# Autodesk Inventor assembly: E-AXIS ASSEMBLY
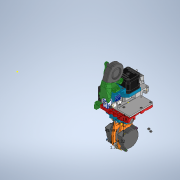
[picture p0: Inventor's stored thumbnail of the model, 180x180]
Saved by Autodesk Inventor 2020 (Build 240168000, 168)
## iProperties
Created: 2019-09-18
Part Number: E-AXIS ASSEMBLY
Document SubType Name: Assembly
Designer: pepd9
Author: pepd9
## Documents named in this file (43)
- C:\DESIGNS\MK3PRO P1\E-Axis\E-AXIS ASSEMBLY.iam
- C:\DESIGNS\MK3PRO P1\COMPONENTS\LM10UU.ipt
- C:\DESIGNS\MK3PRO P1\E-Axis\X-Carriage V1.3.ipt
- C:\DESIGNS\MK3PRO P1\COMPONENTS\M3 Nut.ipt
- C:\DESIGNS\MK3PRO P1\COMPONENTS\SHCS_M3_10.ipt
- C:\DESIGNS\MK3PRO P1\COMPONENTS\SHCS_M3_40.ipt
- C:\DESIGNS\MK3PRO P1\COMPONENTS\NUT_SQUARE_M3.ipt
- C:\DESIGNS\MK3PRO P1\E-Axis\Extruder_stepper_motor.iam
- C:\DESIGNS\MK3PRO P1\COMPONENTS\Bondtech Idler.ipt
- C:\DESIGNS\MK3PRO P1\COMPONENTS\Bondtech Driver.ipt
- C:\DESIGNS\MK3PRO P1\COMPONENTS\SHCS_M3_12.ipt
- C:\DESIGNS\MK3PRO P1\E-Axis\x-Carriage Backplate V1.2.ipt
- C:\DESIGNS\MK3PRO P1\COMPONENTS\SHCS_M3_18.ipt
- C:\DESIGNS\MK3PRO P1\E-Axis\E3D_V6.ipt
- C:\DESIGNS\MK3PRO P1\E-Axis\PINDA_Probe.ipt
- C:\DESIGNS\MK3PRO P1\COMPONENTS\Noctua-NF-A4x10.ipt
- C:\DESIGNS\MK3PRO P1\E-Axis\extruder-cover.ipt
- C:\DESIGNS\MK3PRO P1\E-Axis\Fan Support Front.ipt
- C:\DESIGNS\MK3PRO P1\COMPONENTS\SHCS_M3_8.ipt
- C:\DESIGNS\MK3PRO P1\COMPONENTS\SHCS_M3_20.ipt
- C:\DESIGNS\MK3PRO P1\COMPONENTS\SHCS_M3_14.ipt
- C:\DESIGNS\MK3PRO P1\E-Axis\Endstop Trigger Block.ipt
- C:\DESIGNS\MK3PRO P1\E-Axis\Extruder Back V2.ipt
- C:\DESIGNS\MK3PRO P1\E-Axis\Extruder Idler V2.ipt
- C:\DESIGNS\MK3PRO P1\COMPONENTS\M3 Washer.ipt
- C:\DESIGNS\MK3PRO P1\E-Axis\Front Left FanShrowd V1.0.ipt
- C:\DESIGNS\MK3PRO P1\E-Axis\Left Cable Guide.ipt
- C:\DESIGNS\MK3PRO P1\E-Axis\Teflon Placeholder.ipt
- C:\DESIGNS\MK3PRO P1\COMPONENTS\Small Limit Switch\Small Limit Switch.iam
- C:\DESIGNS\MK3PRO P1\COMPONENTS\SHCS_M3_30.ipt
- C:\DESIGNS\MK3PRO P1\COMPONENTS\SHCS_M3_35.ipt
- C:\DESIGNS\MK3PRO P1\E-Axis\E-Motor Mount P1.1.ipt
- C:\DESIGNS\MK3PRO P1\E-Axis\Extruder Cable Clamp.ipt
- C:\DESIGNS\MK3PRO P1\E-Axis\LimitSwitch Container.ipt
- C:\DESIGNS\MK3PRO P1\E-Axis\LimitSwitch Con Lid.ipt
- C:\DESIGNS\MK3PRO P1\COMPONENTS\FAN_5015_BLOWER.ipt
- C:\DESIGNS\MK3PRO P1\E-Axis\Rear Fan Backplate Mount.ipt
- C:\DESIGNS\MK3PRO P1\E-Axis\Rear Left Fan Cover.ipt
- C:\DESIGNS\MK3PRO P1\E-Axis\Rear Left Fan Mount.ipt
- C:\DESIGNS\MK3PRO P1\E-Axis\Rear Right Fan Mount.ipt
- C:\DESIGNS\MK3PRO P1\E-Axis\Rear Cable Clamp.ipt
- C:\DESIGNS\MK3PRO P1\COMPONENTS\SHCS_M3_25.ipt
- C:\DESIGNS\MK3PRO P1\E-Axis\Rear Cable Clamp1.ipt
## Components (107 placed, 42 different names)
1. LM10UU:1 — Mate:1, Mate:2, Mate:5
2. LM10UU:2 — Mate:1, Mate:3, Mate:6
3. LM10UU:3 — Mate:4, Mate:7
4. X-Carriage V1.3:1 — Mate:2, Mate:3, Mate:4, Mate:5, Mate:6, Mate:7, Flush:1, Mate:8, Mate:9, Mate:10, Mate:11, Mate:12, Mate:13, Mate:14, Mate:15, Mate:16, Mate:17, Mate:18, Mate:19, Mate:20, Mate:21, Mate:22, Mate:23, Mate:24, Mate:25, Mate:26, Mate:28, Mate:30, Mate:44, Mate:46, Mate:47, Mate:48, Mate:49, Mate:73, Mate:74, Mate:75, Mate:76, Mate:77, Mate:78, Mate:79, Mate:97, Mate:98, Mate:152, Mate:153, Mate:154, Mate:155, Mate:156, Mate:157, Mate:158, Mate:159, Mate:160, Mate:161, Mate:162, Mate:163, Mate:164, Mate:165, Mate:166, Mate:170, Angle:4, Mate:186, Mate:188, Mate:247, Mate:248, Mate:249, Mate:250, Mate:251, Mate:252, Mate:254, Mate:255, Flush:18
5. M3 Nut:1 — Mate:11, Mate:25, Mate:26
6. M3 Nut:2 — Mate:12, Mate:23, Mate:24
7. M3 Nut:3 — Mate:13, Mate:28, Mate:158
8. M3 Nut:4 — Mate:15, Mate:17, Mate:18
9. M3 Nut:5 — Mate:10, Mate:21, Mate:22
10. M3 Nut:6 — Mate:14, Mate:30, Mate:159
11. M3 Nut:7 — Mate:16, Mate:19, Mate:20
12. M3 Nut:8
13. M3 Nut:9
14. M3 Nut:10 — Mate:44
15. M3 Nut:11
16. SHCS_M3_10:1 — Mate:46, Mate:49
17. SHCS_M3_10:2 — Mate:47, Mate:48
18. Bondtech Driver:1 — Flush:9
19. SHCS_M3_12:1 — Mate:73, Mate:75
20. SHCS_M3_12:2 — Mate:74, Mate:76
21. x-Carriage Backplate V1.2:1 — Mate:77, Mate:78, Mate:79, Mate:80, Mate:81, Mate:82, Mate:83, Mate:84, Mate:85, Mate:86, Mate:87, Mate:88, Mate:89, Mate:90, Mate:91, Mate:92, Mate:93, Mate:94, Mate:95, Mate:339, Mate:340, Angle:23
22. SHCS_M3_18:1 — Mate:80, Mate:90
23. SHCS_M3_18:2 — Mate:81, Mate:91
24. SHCS_M3_18:3 — Mate:83, Mate:93
25. SHCS_M3_18:4 — Mate:86, Mate:92
26. SHCS_M3_18:5 — Mate:82, Mate:89
27. SHCS_M3_18:6 — Mate:85, Mate:94
28. SHCS_M3_18:7 — Mate:84, Mate:95
29. SHCS_M3_18:8 — Mate:87, Mate:88
30. NUT_SQUARE_M3:3 — Mate:97, Mate:98
31. PINDA_Probe:1 — Mate:220, Mate:221, Flush:11
32. Noctua-NF-A4x10:1 — Mate:138, Mate:139, Mate:144, Mate:145, Mate:195, Angle:6, Mate:225, Mate:226, Mate:260, Mate:261
33. extruder-cover:1 — Mate:192, Mate:193, Mate:194, Mate:195, Angle:6, Mate:231, Angle:11, Mate:256, Mate:262, Mate:263, Mate:264, Mate:300, Mate:301, Mate:302, Mate:320, Angle:22
34. SHCS_M3_18:9 — Mate:138, Mate:145, Mate:194
35. SHCS_M3_18:10 — Mate:139, Mate:144, Mate:235
36. M3 Nut:14 — Mate:153, Mate:155, Mate:156
37. M3 Nut:15 — Mate:152, Mate:154, Mate:157
38. SHCS_M3_14:1 — Mate:161, Mate:162
39. SHCS_M3_14:2 — Mate:160, Mate:163
40. Endstop Trigger Block:1 — Mate:164, Mate:165, Mate:166, Mate:167, Mate:169
41. SHCS_M3_20:3 — Mate:167, Mate:169, Mate:171
42. NUT_SQUARE_M3:6 — Mate:170, Mate:171, Angle:4
43. Extruder Back V2:1 — Mate:173, Mate:179, Mate:184, Mate:185, Mate:186, Mate:188, Mate:196, Mate:197, Angle:7, Flush:10, Mate:217, Mate:220, Mate:221, Mate:233, Mate:234, Angle:12, Mate:244, Mate:272, Angle:15, Mate:280, Mate:282, Mate:293, Mate:296, Mate:297, Mate:298, Angle:19, Mate:299, Angle:20, Flush:18
44. Extruder Idler V2:1 — Mate:173, Mate:177, Mate:178, Mate:183, Mate:198, Mate:199, Mate:200, Mate:229
45. Bondtech Idler:1 — Mate:177, Mate:178, Flush:9
46. M3 Washer:2 — Mate:179, Mate:183
47. E3D_V6:2 — Mate:184, Mate:185, Angle:5, Flush:11, Mate:257, Angle:22
48. Front Left FanShrowd V1.0:1 — Mate:192, Mate:193, Angle:5, Flush:12
49. NUT_SQUARE_M3:7 — Mate:196, Mate:197, Angle:7
50. M3 Washer:3 — Mate:198, Mate:199, Mate:203
51. SHCS_M3_40:2 — Mate:200, Mate:201, Mate:202
52. M3 Washer:4 — Mate:201, Mate:202, Mate:203
53. Left Cable Guide:1 — Flush:10, Mate:245, Mate:276, Mate:277, Angle:17, Mate:289, Mate:290, Angle:18
54. SHCS_M3_8:3 — Mate:244, Mate:245
55. Teflon Placeholder:1 — Mate:217
56. SHCS_M3_14:3 — Mate:225, Mate:226, Mate:232
57. M3 Washer:5 — Mate:229
58. NUT_SQUARE_M3:10 — Mate:231, Mate:232, Angle:11
59. NUT_SQUARE_M3:11 — Mate:234, Mate:235
60. NUT_SQUARE_M3:12 — Mate:233, Angle:12
61. Extruder_stepper_motor:1 [sub-assembly] — Mate:253
62. Small Limit Switch:1 [sub-assembly] — Mate:283, Mate:284, Mate:285, Mate:286
63. SHCS_M3_30:2 — Mate:247, Mate:248
64. SHCS_M3_35:1 — Mate:249, Mate:252, Mate:253, Mate:294
65. SHCS_M3_35:2 — Mate:250, Mate:251
66. SHCS_M3_35:3 — Mate:254, Mate:255, Mate:295
67. E-Motor Mount P1.1:1 — Mate:256, Mate:257, Mate:259, Mate:294, Mate:295
68. SHCS_M3_10:3 — Mate:259
69. SHCS_M3_14:4 — Mate:260, Mate:261, Mate:293
70. SHCS_M3_30:3 — Mate:263, Mate:264
71. SHCS_M3_30:4 — Mate:262, Mate:320
72. SHCS_M3_8:4 — Mate:273, Mate:281
73. NUT_SQUARE_M3:13 — Mate:272, Mate:273, Angle:15
74. Extruder Cable Clamp:1 — Mate:276, Mate:277, Angle:17, Mate:278, Mate:279
75. SHCS_M3_14:5 — Mate:278, Mate:279
76. LimitSwitch Container:1 — Mate:280, Mate:281, Mate:282, Mate:283, Mate:284, Mate:285, Mate:287, Mate:288
77. LimitSwitch Con Lid:1 — Mate:286, Mate:287, Mate:288
78. NUT_SQUARE_M3:14 — Mate:289, Mate:290, Angle:18
79. M3 Nut:16 — Mate:297, Mate:298, Angle:19
80. M3 Nut:17 — Mate:296, Mate:299, Angle:20
81. Fan Support Front:2 — Mate:300, Mate:301, Mate:302, Mate:303, Mate:304, Mate:305
82. FAN_5015_BLOWER:1 — Mate:303, Mate:304, Mate:305, Flush:12
83. FAN_5015_BLOWER:2 — Mate:326, Mate:327, Mate:336, Mate:337, Mate:338, Mate:343, Mate:363
84. Rear Left Fan Cover:1 — Mate:326, Mate:327, Mate:336, Mate:364
85. SHCS_M3_20:4 — Mate:337, Mate:338, Mate:353, Mate:361
86. Rear Left Fan Mount:1 — Mate:341, Mate:342, Mate:343, Mate:346, Angle:26, Mate:353, Mate:358, Mate:359, Mate:360, Angle:28, Angle:29, Mate:365, Mate:372
87. Rear Fan Backplate Mount:1 — Mate:339, Mate:340, Angle:23, Mate:341, Mate:342, Mate:344, Mate:345, Angle:25, Mate:347, Angle:26, Mate:351, Mate:352, Angle:30, Mate:386, Mate:387, Mate:388, Mate:389
88. M3 Nut:18 — Mate:344, Mate:345, Angle:25
89. SHCS_M3_12:3 — Mate:346, Mate:347
90. Rear Right Fan Mount:1 — Mate:349, Mate:350, Mate:351, Mate:354, Mate:355, Mate:356, Angle:30, Mate:366, Mate:367
91. SHCS_M3_12:4 — Mate:349, Mate:350, Mate:352
92. FAN_5015_BLOWER:3 — Mate:354, Mate:355, Mate:356, Mate:368, Mate:369, Mate:370, Mate:371
93. M3 Nut:19
94. M3 Nut:20 — Mate:359, Mate:360, Angle:29
95. M3 Nut:21 — Mate:358, Mate:361, Angle:28
96. SHCS_M3_30:5 — Mate:363, Mate:364, Mate:365, Mate:373
97. Rear Cable Clamp:2 — Mate:366, Mate:367, Angle:31, Mate:374, Mate:376, Mate:377, Mate:378, Mate:379
98. SHCS_M3_25:1 — Mate:368, Mate:371
99. SHCS_M3_20:5 — Mate:369, Mate:370
100. Rear Cable Clamp1:1 — Mate:372, Mate:373, Angle:31
101. SHCS_M3_20:6 — Mate:374, Mate:376
102. SHCS_M3_20:7 — Mate:377
103. SHCS_M3_8:5 — Mate:378, Mate:379
104. SHCS_M3_10:6 — Mate:386, Mate:387
105. SHCS_M3_14:6 — Mate:388, Mate:389
106. M3 Nut:22
107. M3 Nut:23
## Relationships (234: Mate 209, Angle 19, Flush 6)
- Mate:1: LM10UU:1 ↔ LM10UU:2
- Mate:2: LM10UU:1 ↔ X-Carriage V1.3:1
- Mate:3: LM10UU:2 ↔ X-Carriage V1.3:1
- Mate:4: LM10UU:3 ↔ X-Carriage V1.3:1
- Mate:5: LM10UU:1 ↔ X-Carriage V1.3:1
- Mate:6: LM10UU:2 ↔ X-Carriage V1.3:1
- Mate:7: LM10UU:3 ↔ X-Carriage V1.3:1
- Flush:1: X-Carriage V1.3:1
- Mate:8 (-42 mm): X-Carriage V1.3:1
- Mate:9 (14.015 mm): X-Carriage V1.3:1
- Mate:10: X-Carriage V1.3:1 ↔ M3 Nut:5
- Mate:11: X-Carriage V1.3:1 ↔ M3 Nut:1
- Mate:12: X-Carriage V1.3:1 ↔ M3 Nut:2
- Mate:13: X-Carriage V1.3:1 ↔ M3 Nut:3
- Mate:14: X-Carriage V1.3:1 ↔ M3 Nut:6
- Mate:15: X-Carriage V1.3:1 ↔ M3 Nut:4
- Mate:16: X-Carriage V1.3:1 ↔ M3 Nut:7
- Mate:17 (0.085 mm): X-Carriage V1.3:1 ↔ M3 Nut:4
- Mate:18: X-Carriage V1.3:1 ↔ M3 Nut:4
- Mate:19 (0.085 mm): X-Carriage V1.3:1 ↔ M3 Nut:7
- Mate:20: X-Carriage V1.3:1 ↔ M3 Nut:7
- Mate:21 (0.085 mm): X-Carriage V1.3:1 ↔ M3 Nut:5
- Mate:22: X-Carriage V1.3:1 ↔ M3 Nut:5
- Mate:23 (0.085 mm): X-Carriage V1.3:1 ↔ M3 Nut:2
- Mate:24: X-Carriage V1.3:1 ↔ M3 Nut:2
- Mate:25 (0.085 mm): X-Carriage V1.3:1 ↔ M3 Nut:1
- Mate:26: X-Carriage V1.3:1 ↔ M3 Nut:1
- Mate:28: X-Carriage V1.3:1 ↔ M3 Nut:3
- Mate:30: X-Carriage V1.3:1 ↔ M3 Nut:6
- Mate:44: X-Carriage V1.3:1 ↔ M3 Nut:10
- Mate:46: X-Carriage V1.3:1 ↔ SHCS_M3_10:1
- Mate:47: X-Carriage V1.3:1 ↔ SHCS_M3_10:2
- Mate:48: X-Carriage V1.3:1 ↔ SHCS_M3_10:2
- Mate:49: X-Carriage V1.3:1 ↔ SHCS_M3_10:1
- Mate:73: X-Carriage V1.3:1 ↔ SHCS_M3_12:1
- Mate:74: X-Carriage V1.3:1 ↔ SHCS_M3_12:2
- Mate:75: X-Carriage V1.3:1 ↔ SHCS_M3_12:1
- Mate:76: X-Carriage V1.3:1 ↔ SHCS_M3_12:2
- Mate:77: X-Carriage V1.3:1 ↔ x-Carriage Backplate V1.2:1
- Mate:78: X-Carriage V1.3:1 ↔ x-Carriage Backplate V1.2:1
- Mate:79: X-Carriage V1.3:1 ↔ x-Carriage Backplate V1.2:1
- Mate:80: x-Carriage Backplate V1.2:1 ↔ SHCS_M3_18:1
- Mate:81: x-Carriage Backplate V1.2:1 ↔ SHCS_M3_18:2
- Mate:82: x-Carriage Backplate V1.2:1 ↔ SHCS_M3_18:5
- Mate:83: x-Carriage Backplate V1.2:1 ↔ SHCS_M3_18:3
- Mate:84: x-Carriage Backplate V1.2:1 ↔ SHCS_M3_18:7
- Mate:85: x-Carriage Backplate V1.2:1 ↔ SHCS_M3_18:6
- Mate:86: x-Carriage Backplate V1.2:1 ↔ SHCS_M3_18:4
- Mate:87: x-Carriage Backplate V1.2:1 ↔ SHCS_M3_18:8
- Mate:88: x-Carriage Backplate V1.2:1 ↔ SHCS_M3_18:8
- Mate:89: x-Carriage Backplate V1.2:1 ↔ SHCS_M3_18:5
- Mate:90: x-Carriage Backplate V1.2:1 ↔ SHCS_M3_18:1
- Mate:91: x-Carriage Backplate V1.2:1 ↔ SHCS_M3_18:2
- Mate:92: x-Carriage Backplate V1.2:1 ↔ SHCS_M3_18:4
- Mate:93: x-Carriage Backplate V1.2:1 ↔ SHCS_M3_18:3
- Mate:94: x-Carriage Backplate V1.2:1 ↔ SHCS_M3_18:6
- Mate:95: x-Carriage Backplate V1.2:1 ↔ SHCS_M3_18:7
- Mate:97: X-Carriage V1.3:1 ↔ NUT_SQUARE_M3:3
- Mate:98: X-Carriage V1.3:1 ↔ NUT_SQUARE_M3:3
- Mate:138: Noctua-NF-A4x10:1 ↔ SHCS_M3_18:9
- Mate:139: Noctua-NF-A4x10:1 ↔ SHCS_M3_18:10
- Mate:144: Noctua-NF-A4x10:1 ↔ SHCS_M3_18:10
- Mate:145: Noctua-NF-A4x10:1 ↔ SHCS_M3_18:9
- Mate:152: X-Carriage V1.3:1 ↔ M3 Nut:15
- Mate:153: X-Carriage V1.3:1 ↔ M3 Nut:14
- Mate:154: X-Carriage V1.3:1 ↔ M3 Nut:15
- Mate:155: X-Carriage V1.3:1 ↔ M3 Nut:14
- Mate:156 (0.085 mm): X-Carriage V1.3:1 ↔ M3 Nut:14
- Mate:157 (0.085 mm): X-Carriage V1.3:1 ↔ M3 Nut:15
- Mate:158: X-Carriage V1.3:1 ↔ M3 Nut:3
- Mate:159: X-Carriage V1.3:1 ↔ M3 Nut:6
- Mate:160: X-Carriage V1.3:1 ↔ SHCS_M3_14:2
- Mate:161: X-Carriage V1.3:1 ↔ SHCS_M3_14:1
- Mate:162 (10 mm): X-Carriage V1.3:1 ↔ SHCS_M3_14:1
- Mate:163 (10 mm): X-Carriage V1.3:1 ↔ SHCS_M3_14:2
- Mate:164: X-Carriage V1.3:1 ↔ Endstop Trigger Block:1
- Mate:165: X-Carriage V1.3:1 ↔ Endstop Trigger Block:1
- Mate:166: X-Carriage V1.3:1 ↔ Endstop Trigger Block:1
- Mate:167: Endstop Trigger Block:1 ↔ SHCS_M3_20:3
- Mate:169: Endstop Trigger Block:1 ↔ SHCS_M3_20:3
- Mate:170: X-Carriage V1.3:1 ↔ NUT_SQUARE_M3:6
- Mate:171: SHCS_M3_20:3 ↔ NUT_SQUARE_M3:6
- Angle:4 (0 deg): X-Carriage V1.3:1 ↔ NUT_SQUARE_M3:6
- Mate:173: Extruder Back V2:1 ↔ Extruder Idler V2:1
- Mate:177: Extruder Idler V2:1 ↔ Bondtech Idler:1
- Mate:178 (0.3 mm): Extruder Idler V2:1 ↔ Bondtech Idler:1
- Mate:179: Extruder Back V2:1 ↔ M3 Washer:2
- Mate:183: Extruder Idler V2:1 ↔ M3 Washer:2
- Mate:184: Extruder Back V2:1 ↔ E3D_V6:2
- Mate:185: Extruder Back V2:1 ↔ E3D_V6:2
- Mate:186: X-Carriage V1.3:1 ↔ Extruder Back V2:1
- Flush:9: Bondtech Driver:1 ↔ Bondtech Idler:1
- Mate:188: X-Carriage V1.3:1 ↔ Extruder Back V2:1
- Mate:192: extruder-cover:1 ↔ Front Left FanShrowd V1.0:1
- Mate:193: extruder-cover:1 ↔ Front Left FanShrowd V1.0:1
- Angle:5 (0 deg): E3D_V6:2 ↔ Front Left FanShrowd V1.0:1
- Mate:194: extruder-cover:1 ↔ SHCS_M3_18:9
- Mate:195: Noctua-NF-A4x10:1 ↔ extruder-cover:1
- Angle:6 (0 deg): Noctua-NF-A4x10:1 ↔ extruder-cover:1
- Mate:196: Extruder Back V2:1 ↔ NUT_SQUARE_M3:7
- Mate:197: Extruder Back V2:1 ↔ NUT_SQUARE_M3:7
- Angle:7 (0 deg): Extruder Back V2:1 ↔ NUT_SQUARE_M3:7
- Mate:198: Extruder Idler V2:1 ↔ M3 Washer:3
- Mate:199: Extruder Idler V2:1 ↔ M3 Washer:3
- Mate:200: Extruder Idler V2:1 ↔ SHCS_M3_40:2
- Mate:201: SHCS_M3_40:2 ↔ M3 Washer:4
- Mate:202: SHCS_M3_40:2 ↔ M3 Washer:4
- Mate:203 (13 mm): M3 Washer:3 ↔ M3 Washer:4
- Flush:10: Extruder Back V2:1 ↔ Left Cable Guide:1
- Mate:217: Extruder Back V2:1 ↔ Teflon Placeholder:1
- Mate:220 (9 mm): PINDA_Probe:1 ↔ Extruder Back V2:1
- Mate:221 (-5 mm): PINDA_Probe:1 ↔ Extruder Back V2:1
- Flush:11 (2 mm): PINDA_Probe:1 ↔ E3D_V6:2
- Mate:225: Noctua-NF-A4x10:1 ↔ SHCS_M3_14:3
- Mate:226: Noctua-NF-A4x10:1 ↔ SHCS_M3_14:3
- Mate:229: Extruder Idler V2:1 ↔ M3 Washer:5
- Mate:231: extruder-cover:1 ↔ NUT_SQUARE_M3:10
- Mate:232: SHCS_M3_14:3 ↔ NUT_SQUARE_M3:10
- Angle:11 (0 deg): extruder-cover:1 ↔ NUT_SQUARE_M3:10
- Mate:233: Extruder Back V2:1 ↔ NUT_SQUARE_M3:12
- Mate:234: Extruder Back V2:1 ↔ NUT_SQUARE_M3:11
- Mate:235: SHCS_M3_18:10 ↔ NUT_SQUARE_M3:11
- Angle:12 (0 deg): Extruder Back V2:1 ↔ NUT_SQUARE_M3:12
- Mate:244: Extruder Back V2:1 ↔ SHCS_M3_8:3
- Mate:245: Left Cable Guide:1 ↔ SHCS_M3_8:3
- Mate:247: X-Carriage V1.3:1 ↔ SHCS_M3_30:2
- Mate:248: X-Carriage V1.3:1 ↔ SHCS_M3_30:2
- Mate:249: X-Carriage V1.3:1 ↔ SHCS_M3_35:1
- Mate:250: X-Carriage V1.3:1 ↔ SHCS_M3_35:2
- Mate:251: X-Carriage V1.3:1 ↔ SHCS_M3_35:2
- Mate:252: X-Carriage V1.3:1 ↔ SHCS_M3_35:1
- Mate:253: Extruder_stepper_motor:1 ↔ SHCS_M3_35:1
- Mate:254: X-Carriage V1.3:1 ↔ SHCS_M3_35:3
- Mate:255: X-Carriage V1.3:1 ↔ SHCS_M3_35:3
- Mate:256: extruder-cover:1 ↔ E-Motor Mount P1.1:1
- Mate:257: E3D_V6:2 ↔ E-Motor Mount P1.1:1
- Mate:259: E-Motor Mount P1.1:1 ↔ SHCS_M3_10:3
- Mate:260: Noctua-NF-A4x10:1 ↔ SHCS_M3_14:4
- Mate:261: Noctua-NF-A4x10:1 ↔ SHCS_M3_14:4
- Mate:262: extruder-cover:1 ↔ SHCS_M3_30:4
- Mate:263: extruder-cover:1 ↔ SHCS_M3_30:3
- Mate:264: extruder-cover:1 ↔ SHCS_M3_30:3
- Mate:272: Extruder Back V2:1 ↔ NUT_SQUARE_M3:13
- Mate:273: SHCS_M3_8:4 ↔ NUT_SQUARE_M3:13
- Angle:15 (0 deg): Extruder Back V2:1 ↔ NUT_SQUARE_M3:13
- Mate:276: Left Cable Guide:1 ↔ Extruder Cable Clamp:1
- Mate:277: Left Cable Guide:1 ↔ Extruder Cable Clamp:1
- Angle:17 (0 deg): Left Cable Guide:1 ↔ Extruder Cable Clamp:1
- Mate:278: Extruder Cable Clamp:1 ↔ SHCS_M3_14:5
- Mate:279: Extruder Cable Clamp:1 ↔ SHCS_M3_14:5
- Mate:280: Extruder Back V2:1 ↔ LimitSwitch Container:1
- Mate:281: SHCS_M3_8:4 ↔ LimitSwitch Container:1
- Mate:282: Extruder Back V2:1 ↔ LimitSwitch Container:1
- Mate:283: Small Limit Switch:1 ↔ LimitSwitch Container:1
- Mate:284: Small Limit Switch:1 ↔ LimitSwitch Container:1
- Mate:285: Small Limit Switch:1 ↔ LimitSwitch Container:1
- Mate:286: Small Limit Switch:1 ↔ LimitSwitch Con Lid:1
- Mate:287: LimitSwitch Container:1 ↔ LimitSwitch Con Lid:1
- Mate:288: LimitSwitch Container:1 ↔ LimitSwitch Con Lid:1
- Mate:289: Left Cable Guide:1 ↔ NUT_SQUARE_M3:14
- Mate:290: Left Cable Guide:1 ↔ NUT_SQUARE_M3:14
- Angle:18 (0 deg): Left Cable Guide:1 ↔ NUT_SQUARE_M3:14
- Mate:293: Extruder Back V2:1 ↔ SHCS_M3_14:4
- Mate:294: SHCS_M3_35:1 ↔ E-Motor Mount P1.1:1
- Mate:295: SHCS_M3_35:3 ↔ E-Motor Mount P1.1:1
- Mate:296: Extruder Back V2:1 ↔ M3 Nut:17
- Mate:297: Extruder Back V2:1 ↔ M3 Nut:16
- Mate:298: Extruder Back V2:1 ↔ M3 Nut:16
- Angle:19 (0 deg): Extruder Back V2:1 ↔ M3 Nut:16
- Mate:299: Extruder Back V2:1 ↔ M3 Nut:17
- Angle:20 (0 deg): Extruder Back V2:1 ↔ M3 Nut:17
- Mate:300: extruder-cover:1 ↔ Fan Support Front:2
- Mate:301: extruder-cover:1 ↔ Fan Support Front:2
- Mate:302: extruder-cover:1 ↔ Fan Support Front:2
- Mate:303: Fan Support Front:2 ↔ FAN_5015_BLOWER:1
- Mate:304: Fan Support Front:2 ↔ FAN_5015_BLOWER:1
- Mate:305: Fan Support Front:2 ↔ FAN_5015_BLOWER:1
- Flush:12: Front Left FanShrowd V1.0:1 ↔ FAN_5015_BLOWER:1
- Mate:320: extruder-cover:1 ↔ SHCS_M3_30:4
- Flush:18: X-Carriage V1.3:1 ↔ Extruder Back V2:1
- Mate:326: FAN_5015_BLOWER:2 ↔ Rear Left Fan Cover:1
- Mate:327: FAN_5015_BLOWER:2 ↔ Rear Left Fan Cover:1
- Angle:22 (0 deg): extruder-cover:1 ↔ E3D_V6:2
- Mate:336: FAN_5015_BLOWER:2 ↔ Rear Left Fan Cover:1
- Mate:337: FAN_5015_BLOWER:2 ↔ SHCS_M3_20:4
- Mate:338: FAN_5015_BLOWER:2 ↔ SHCS_M3_20:4
- Mate:339: x-Carriage Backplate V1.2:1 ↔ Rear Fan Backplate Mount:1
- Mate:340: x-Carriage Backplate V1.2:1 ↔ Rear Fan Backplate Mount:1
- Angle:23 (0 deg): x-Carriage Backplate V1.2:1 ↔ Rear Fan Backplate Mount:1
- Mate:341: Rear Left Fan Mount:1 ↔ Rear Fan Backplate Mount:1
- Mate:342: Rear Left Fan Mount:1 ↔ Rear Fan Backplate Mount:1
- Mate:343: FAN_5015_BLOWER:2 ↔ Rear Left Fan Mount:1
- Mate:344: Rear Fan Backplate Mount:1 ↔ M3 Nut:18
- Mate:345: Rear Fan Backplate Mount:1 ↔ M3 Nut:18
- Angle:25 (0 deg): Rear Fan Backplate Mount:1 ↔ M3 Nut:18
- Mate:346: Rear Left Fan Mount:1 ↔ SHCS_M3_12:3
- Mate:347 (6 mm): Rear Fan Backplate Mount:1 ↔ SHCS_M3_12:3
- Angle:26 (0 deg): Rear Left Fan Mount:1 ↔ Rear Fan Backplate Mount:1
- Mate:349: Rear Right Fan Mount:1 ↔ SHCS_M3_12:4
- Mate:350: Rear Right Fan Mount:1 ↔ SHCS_M3_12:4
- Mate:351: Rear Fan Backplate Mount:1 ↔ Rear Right Fan Mount:1
- Mate:352: Rear Fan Backplate Mount:1 ↔ SHCS_M3_12:4
- Mate:353: SHCS_M3_20:4 ↔ Rear Left Fan Mount:1
- Mate:354: Rear Right Fan Mount:1 ↔ FAN_5015_BLOWER:3
- Mate:355: Rear Right Fan Mount:1 ↔ FAN_5015_BLOWER:3
- Mate:356: Rear Right Fan Mount:1 ↔ FAN_5015_BLOWER:3
- Mate:358: Rear Left Fan Mount:1 ↔ M3 Nut:21
- Mate:359: Rear Left Fan Mount:1 ↔ M3 Nut:20
- Mate:360: Rear Left Fan Mount:1 ↔ M3 Nut:20
- Mate:361: SHCS_M3_20:4 ↔ M3 Nut:21
- Angle:28 (0 deg): Rear Left Fan Mount:1 ↔ M3 Nut:21
- Angle:29 (0 deg): Rear Left Fan Mount:1 ↔ M3 Nut:20
- Mate:363: FAN_5015_BLOWER:2 ↔ SHCS_M3_30:5
- Mate:364: Rear Left Fan Cover:1 ↔ SHCS_M3_30:5
- Angle:30 (0 deg): Rear Fan Backplate Mount:1 ↔ Rear Right Fan Mount:1
- Mate:365: Rear Left Fan Mount:1 ↔ SHCS_M3_30:5
- Mate:366: Rear Right Fan Mount:1 ↔ Rear Cable Clamp:2
- Mate:367: Rear Right Fan Mount:1 ↔ Rear Cable Clamp:2
- Mate:368: FAN_5015_BLOWER:3 ↔ SHCS_M3_25:1
- Mate:369: FAN_5015_BLOWER:3 ↔ SHCS_M3_20:5
- Mate:370: FAN_5015_BLOWER:3 ↔ SHCS_M3_20:5
- Mate:371: FAN_5015_BLOWER:3 ↔ SHCS_M3_25:1
- Mate:372: Rear Left Fan Mount:1 ↔ Rear Cable Clamp1:1
- Mate:373: SHCS_M3_30:5 ↔ Rear Cable Clamp1:1
- Angle:31 (0 deg): Rear Cable Clamp:2 ↔ Rear Cable Clamp1:1
- Mate:374: Rear Cable Clamp:2 ↔ SHCS_M3_20:6
- Mate:376: Rear Cable Clamp:2 ↔ SHCS_M3_20:6
- Mate:377: Rear Cable Clamp:2 ↔ SHCS_M3_20:7
- Mate:378: Rear Cable Clamp:2 ↔ SHCS_M3_8:5
- Mate:379: Rear Cable Clamp:2 ↔ SHCS_M3_8:5
- Mate:386: Rear Fan Backplate Mount:1 ↔ SHCS_M3_10:6
- Mate:387: Rear Fan Backplate Mount:1 ↔ SHCS_M3_10:6
- Mate:388: Rear Fan Backplate Mount:1 ↔ SHCS_M3_14:6
- Mate:389: Rear Fan Backplate Mount:1 ↔ SHCS_M3_14:6
